# Autodesk Inventor assembly: ensamblado
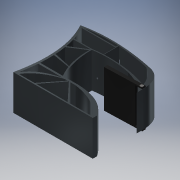
[picture p0: Inventor's stored thumbnail of the model, 180x180]
Saved by Autodesk Inventor 2018 (Build 220112000, 112)
## iProperties
Created: 2018-01-13
Part Number: ensamblado
Document SubType Name: Assembly
Designer: mokuz
Author: mokuz
## Documents named in this file (4)
- D:\proyectos\silla_dani\ensamblado.iam
- D:\proyectos\silla_dani\silla.ipt
- D:\proyectos\silla_dani\eje.ipt
- D:\proyectos\silla_dani\mesa.ipt
## Components (3 placed, 3 different names)
1. silla:1 — Insert:1
2. eje:1 — Insert:1, Insert:2
3. mesa:1 — Insert:2
## Relationships (2: Insert 2)
- Insert:1 (-30 mm): silla:1 ↔ eje:1
- Insert:2: eje:1 ↔ mesa:1
